# Autodesk Inventor assembly: Prueba3
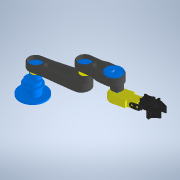
[picture p0: Inventor's stored thumbnail of the model, 180x180]
Saved by Autodesk Inventor 2021 (Build 250183000, 183)
## iProperties
Created: 2022-04-22
Part Number: Prueba3
Document SubType Name: Assembly
Designer: Alcatraz
Author: Alcatraz
## Documents named in this file (5)
- F:\Tesis\TESIS\Matlab\Pruebas\Prueba3_Simulacion1\Prueba3.iam
- F:\Tesis\TESIS\Base_Prueba1.iam
- F:\Tesis\TESIS\Matlab\Pruebas\Prueba3_Simulacion1\Eslabon1.ipt
- F:\Tesis\TESIS\Matlab\Pruebas\Prueba3_Simulacion1\Eslabon2.ipt
- F:\Tesis\TESIS\Matlab\Pruebas\Prueba3_Simulacion1\Eslabon3.ipt
## Components (4 placed, 4 different names)
1. Base_Prueba1:1 [sub-assembly] — De rotación:1
2. Eslabon1:1 — De rotación:1, De rotación:2
3. Eslabon2:1 — De rotación:2, De rotación:3
4. Eslabon3:1 — De rotación:3
## Relationships (3: RevoluteJoint 3)
- De rotación:1 [RevoluteJoint]: Base_Prueba1:1 ↔ Eslabon1:1
- De rotación:2 [RevoluteJoint]: Eslabon1:1 ↔ Eslabon2:1
- De rotación:3 [RevoluteJoint]: Eslabon2:1 ↔ Eslabon3:1
